# Autodesk Inventor assembly: flipper_tensioner
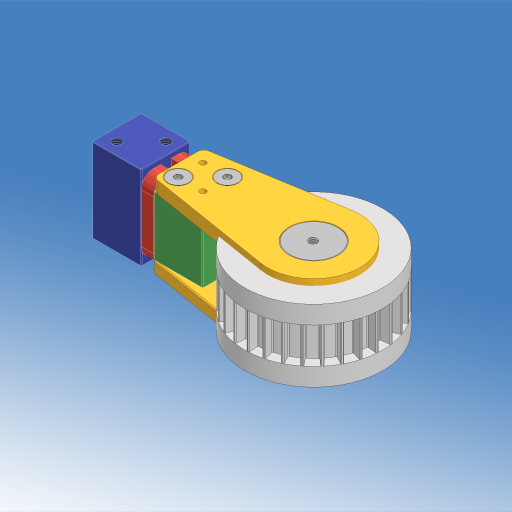
[picture p0: Inventor's stored thumbnail of the model, 512x512]
Saved by Autodesk Inventor 2024 (Build 280153000, 153)
## iProperties
Created: 2023-02-28
Part Number: flipper_tensioner
Document SubType Name: Assembly
Designer: ralph
Author: ralph
## Documents named in this file (11)
- C:\Users\seene\OneDrive\SBRT\Robocup Rescue\Drive\v1\TANK flipper\flipper_tensioner _belt.iam
- C:\Users\seene\OneDrive\SBRT\Robocup Rescue\Drive\v1\TANK flipper\Idler Shaft.ipt
- C:\Users\seene\OneDrive\SBRT\Robocup Rescue\Drive\v1\TANK flipper\tensioner anchor block.ipt
- C:\Users\seene\OneDrive\SBRT\Robocup Rescue\Drive\v1\TANK flipper\tensioner inside plate.ipt
- C:\Users\seene\OneDrive\SBRT\Robocup Rescue\Drive\v1\TANK flipper\tensioner mobile block.ipt
- C:\Users\seene\OneDrive\SBRT\Robocup Rescue\Drive\v1\TANK flipper\tensioner outside plate.ipt
- C:\Users\seene\OneDrive\SBRT\Robocup Rescue\Drive\v1\TANK flipper\tensioner spacer.ipt
- C:\Users\seene\OneDrive\SBRT\Robocup Rescue\Drive\v1\TANK flipper\91253A245_Black-Oxide Alloy Steel Hex Drive Flat Head Screw v1.ipt
- C:\Users\seene\OneDrive\SBRT\Robocup Rescue\Drive\v1\TANK flipper\90128A229_Zinc-Plated Alloy Steel Socket Head Screw (1) v1.ipt
- C:\Users\seene\OneDrive\SBRT\Robocup Rescue\Drive\v1\TANK flipper\VTR-015_pulley.ipt
- C:\Users\seene\OneDrive\SBRT\Robocup Rescue\Drive\v1\TANK flipper\2868T199_High-Load Oil-Embedded 863 Sleeve Bearing (1) v2.ipt
## Components (14 placed, 10 different names)
1. Idler Shaft:1 — Mate:13, Flush:1, Mate:21
2. tensioner anchor block:1 — Mate:9, Mate:10, Mate:19, Mate:22
3. tensioner inside plate:1 — Mate:1, Mate:2, Mate:3, Mate:4, Mate:5, Mate:14, Flush:3, Mate:15, Flush:4
4. tensioner mobile block:1 — Mate:1, Mate:2, Mate:3, Mate:6, Mate:7, Mate:8, Mate:9, Mate:10, Mate:11, Mate:12
5. tensioner outside plate:1 — Mate:4, Mate:5, Mate:6, Mate:13, Flush:1, Mate:16, Mate:17, Flush:5, Flush:6, Flush:7
6. tensioner spacer:1 — Mate:7, Mate:8, Mate:22
7. 91253A245_Black-Oxide Alloy Steel Hex Drive Flat Head Screw v1:2 — Mate:15, Flush:4
8. 91253A245_Black-Oxide Alloy Steel Hex Drive Flat Head Screw v1:3 — Mate:14, Flush:3
9. 91253A245_Black-Oxide Alloy Steel Hex Drive Flat Head Screw v1:4 — Mate:17, Flush:6
10. 91253A245_Black-Oxide Alloy Steel Hex Drive Flat Head Screw v1:5 — Mate:16, Flush:5
11. 90128A229_Zinc-Plated Alloy Steel Socket Head Screw (1) v1:1 — Mate:11, Flush:2, Mate:19
12. 90128A229_Zinc-Plated Alloy Steel Socket Head Screw (1) v1:2 — Mate:12, Flush:2
13. VTR-015_pulley:1 — Mate:20, Flush:7
14. 2868T199_High-Load Oil-Embedded 863 Sleeve Bearing (1) v2:1 — Mate:20, Mate:21
## Relationships (28: Mate 21, Flush 7)
- Mate:1: tensioner inside plate:1 ↔ tensioner mobile block:1
- Mate:2: tensioner inside plate:1 ↔ tensioner mobile block:1
- Mate:3: tensioner inside plate:1 ↔ tensioner mobile block:1
- Mate:4: tensioner inside plate:1 ↔ tensioner outside plate:1
- Mate:5: tensioner inside plate:1 ↔ tensioner outside plate:1
- Mate:6: tensioner mobile block:1 ↔ tensioner outside plate:1
- Mate:7: tensioner mobile block:1 ↔ tensioner spacer:1
- Mate:8: tensioner mobile block:1 ↔ tensioner spacer:1
- Mate:9: tensioner anchor block:1 ↔ tensioner mobile block:1
- Mate:10: tensioner anchor block:1 ↔ tensioner mobile block:1
- Mate:11: tensioner mobile block:1 ↔ 90128A229_Zinc-Plated Alloy Steel Socket Head Screw (1) v1:1
- Mate:12: tensioner mobile block:1 ↔ 90128A229_Zinc-Plated Alloy Steel Socket Head Screw (1) v1:2
- Mate:13: Idler Shaft:1 ↔ tensioner outside plate:1
- Flush:1: Idler Shaft:1 ↔ tensioner outside plate:1
- Flush:2: 90128A229_Zinc-Plated Alloy Steel Socket Head Screw (1) v1:1 ↔ 90128A229_Zinc-Plated Alloy Steel Socket Head Screw (1) v1:2
- Mate:14: tensioner inside plate:1 ↔ 91253A245_Black-Oxide Alloy Steel Hex Drive Flat Head Screw v1:3
- Flush:3: tensioner inside plate:1 ↔ 91253A245_Black-Oxide Alloy Steel Hex Drive Flat Head Screw v1:3
- Mate:15: tensioner inside plate:1 ↔ 91253A245_Black-Oxide Alloy Steel Hex Drive Flat Head Screw v1:2
- Flush:4: tensioner inside plate:1 ↔ 91253A245_Black-Oxide Alloy Steel Hex Drive Flat Head Screw v1:2
- Mate:16: tensioner outside plate:1 ↔ 91253A245_Black-Oxide Alloy Steel Hex Drive Flat Head Screw v1:5
- Mate:17: tensioner outside plate:1 ↔ 91253A245_Black-Oxide Alloy Steel Hex Drive Flat Head Screw v1:4
- Flush:5: tensioner outside plate:1 ↔ 91253A245_Black-Oxide Alloy Steel Hex Drive Flat Head Screw v1:5
- Flush:6: tensioner outside plate:1 ↔ 91253A245_Black-Oxide Alloy Steel Hex Drive Flat Head Screw v1:4
- Mate:19: tensioner anchor block:1 ↔ 90128A229_Zinc-Plated Alloy Steel Socket Head Screw (1) v1:1
- Mate:20: VTR-015_pulley:1 ↔ 2868T199_High-Load Oil-Embedded 863 Sleeve Bearing (1) v2:1
- Mate:21: Idler Shaft:1 ↔ 2868T199_High-Load Oil-Embedded 863 Sleeve Bearing (1) v2:1
- Flush:7 (-3.175 mm): tensioner outside plate:1 ↔ VTR-015_pulley:1
- Mate:22: tensioner anchor block:1 ↔ tensioner spacer:1
